# Autodesk Inventor assembly: Assembled_Case
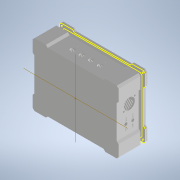
[picture p0: Inventor's stored thumbnail of the model, 180x180]
Saved by Autodesk Inventor 2021.1 (Build 251245000, 245)
## iProperties
Created: 2020-06-02
Part Number: Assembled_Case
Document SubType Name: Assembly
Designer: Alex
Author: Alex
## Documents named in this file (3)
- C:\Users\Alex\3D Objects\Inventor\Omnitrigger_Models\Assembled_Case.iam
- C:\Users\Alex\3D Objects\Inventor\Omnitrigger_Models\Case.ipt
- C:\Users\Alex\3D Objects\Inventor\Omnitrigger_Models\Lid.ipt
## Components (2 placed, 2 different names)
1. Case:1 — Flush:1
2. Lid:1 — Flush:2
## Relationships (2: Flush 2)
- Flush:1 (10 mm): Case:1
- Flush:2: Lid:1
